# Autodesk Inventor assembly: ABD_Slider_Set
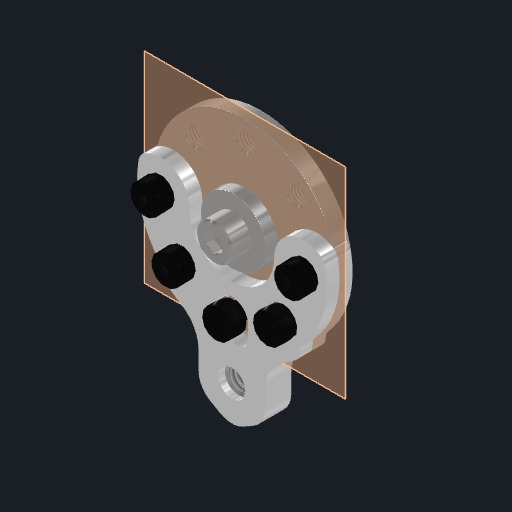
[picture p0: Inventor's stored thumbnail of the model, 512x512]
Saved by Autodesk Inventor 2024 (Build 280153000, 153)
## iProperties
Created: 2024-02-15
Part Number: ABD_Slider_Set
Document SubType Name: Assembly
Designer: ASUS
Author: ASUS
## Documents named in this file (6)
- C:\Users\ASUS\Desktop\Anti_Backlash_Structure_OP\v3_Frame\ABD_Slider_Set_v3.iam
- C:\Users\ASUS\Desktop\Anti_Backlash_Structure_OP\ROBOTIS(Inventor 2024 ver.)\HORN\64-106Horn.ipt
- C:\Users\ASUS\Desktop\Anti_Backlash_Structure_OP\MISUMI\CSH-STN-M3-10_203.ipt
- C:\Users\ASUS\Desktop\Anti_Backlash_Structure_OP\MISUMI\4mm_ABD_set.iam
- C:\Users\ASUS\Desktop\Anti_Backlash_Structure_OP\v3_Frame\Slider_crank_horn_v3.ipt
- C:\Users\ASUS\Documents\Inventor\Content Center Files\R2024\ko-KR\ANSI B 18.2.4.1 M(1)\ANSI B 18.2.4.1 M - M4 x 0.7Style 1.ipt
## Components (5 placed, 5 different names)
1. 64-106Horn:1 — 삽입:3, 삽입:4, 메이트:3
2. CSH-STN-M3-10_203:1 — 삽입:3
3. 4mm_ABD_set:1 [sub-assembly] — 메이트:1, 메이트:2, 메이트:3, 삽입:5
4. 6각 너트 미터 M4 x 0.7:1 — 각도:1
5. Slider_crank_horn_v3:1 — 삽입:4, 메이트:1, 메이트:2, 삽입:5
## Relationships (7: Insert 3, Mate 3, Angle 1)
- 삽입:3 [Insert]: 64-106Horn:1 ↔ CSH-STN-M3-10_203:1
- 각도:1 [Angle] (0 deg): 6각 너트 미터 M4 x 0.7:1
- 삽입:4 [Insert]: 64-106Horn:1 ↔ Slider_crank_horn_v3:1
- 메이트:1 [Mate]: 4mm_ABD_set:1 ↔ Slider_crank_horn_v3:1
- 메이트:2 [Mate]: 4mm_ABD_set:1 ↔ Slider_crank_horn_v3:1
- 메이트:3 [Mate]: 64-106Horn:1 ↔ 4mm_ABD_set:1
- 삽입:5 [Insert]: 4mm_ABD_set:1 ↔ Slider_crank_horn_v3:1
